# Autodesk Inventor assembly: ЛЦМК000002.00.02.00.00.00 Второй вариант крепления.ipt
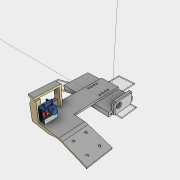
[picture p0: Inventor's stored thumbnail of the model, 180x180]
Saved by Autodesk Inventor 2021.2 (Build 252289000, 289)
## iProperties
Created: 2025-11-08
Part Number: ЛЦМК000002.00.02.00.00.00 Второй вариант крепления.ipt
Document SubType Name: Assembly
Designer: Захаров
Author: Захаров
## Documents named in this file (6)
- C:\Users\User\Documents\CaseARHead1\ЛЦМК000002.00.02.00.00.00 Второй вариант крепления.ipt.iam
- C:\Users\User\Documents\CaseARHead1\ЛЦМК000002.00.00.00.00.08-01.ipt
- C:\Users\User\Documents\CaseARHead1\ЛЦМК000002.00.00.00.00.15.ipt
- C:\Users\User\Documents\CaseARHead1\ЛЦМК000002.00.00.00.00.18.ipt
- C:\Users\User\Documents\CaseARHead1\ЛЦМК000002.00.00.00.00.06-05.ipt
- C:\Users\User\Documents\CaseARHead1\Сборка1.iam
## Components (5 placed, 5 different names)
1. ЛЦМК000002.00.00.00.00.08-01:1 — Заподлицо:1, Совмещение:2, Совмещение:3, Совмещение:4
2. ЛЦМК000002.00.00.00.00.15:1 — Заподлицо:1, Заподлицо:2, Заподлицо:3, Совмещение:1, Совмещение:2, Совмещение:3
3. ЛЦМК000002.00.00.00.00.18:1 — Заподлицо:2, Заподлицо:3, Совмещение:1, Совмещение:7, Заподлицо:4
4. ЛЦМК000002.00.00.00.00.06-05:1 — Совмещение:4, Совмещение:5, Совмещение:6, Совмещение:7, Заподлицо:4
5. Сборка1:1 [sub-assembly] — Совмещение:5, Совмещение:6
## Relationships (11: Mate 7, Flush 4)
- Заподлицо:1 [Flush]: ЛЦМК000002.00.00.00.00.08-01:1 ↔ ЛЦМК000002.00.00.00.00.15:1
- Заподлицо:2 [Flush]: ЛЦМК000002.00.00.00.00.15:1 ↔ ЛЦМК000002.00.00.00.00.18:1
- Заподлицо:3 [Flush]: ЛЦМК000002.00.00.00.00.15:1 ↔ ЛЦМК000002.00.00.00.00.18:1
- Совмещение:1 [Mate] (-2 mm): ЛЦМК000002.00.00.00.00.15:1 ↔ ЛЦМК000002.00.00.00.00.18:1
- Совмещение:2 [Mate]: ЛЦМК000002.00.00.00.00.08-01:1 ↔ ЛЦМК000002.00.00.00.00.15:1
- Совмещение:3 [Mate]: ЛЦМК000002.00.00.00.00.08-01:1 ↔ ЛЦМК000002.00.00.00.00.15:1
- Совмещение:4 [Mate]: ЛЦМК000002.00.00.00.00.08-01:1 ↔ ЛЦМК000002.00.00.00.00.06-05:1
- Совмещение:5 [Mate]: ЛЦМК000002.00.00.00.00.06-05:1 ↔ Сборка1:1
- Совмещение:6 [Mate]: ЛЦМК000002.00.00.00.00.06-05:1 ↔ Сборка1:1
- Совмещение:7 [Mate]: ЛЦМК000002.00.00.00.00.18:1 ↔ ЛЦМК000002.00.00.00.00.06-05:1
- Заподлицо:4 [Flush]: ЛЦМК000002.00.00.00.00.18:1 ↔ ЛЦМК000002.00.00.00.00.06-05:1
